# Autodesk Inventor assembly: LightBracketAssembly
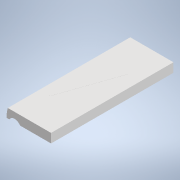
[picture p0: Inventor's stored thumbnail of the model, 180x180]
Saved by Autodesk Inventor 2021.2 (Build 252289000, 289)
## iProperties
Created: 2021-02-05
Part Number: LightBracketAssembly
Document SubType Name: Assembly
Designer: robst
Author: robst
## Documents named in this file (3)
- C:\git\CAD-Development\robSteele\HouseProjects\TrailerProjects\LightBracketAssembly.iam
- C:\git\CAD-Development\robSteele\HouseProjects\TrailerProjects\ketchenLightBracketV02-leftSide.ipt
- C:\git\CAD-Development\robSteele\HouseProjects\TrailerProjects\ketchenLightBracketV02-rightSide.ipt
## Components (2 placed, 2 different names)
1. ketchenLightBracketV02-leftSide:1 — Flush:1, Flush:2, Mate:1
2. ketchenLightBracketV02-rightSide:1 — Flush:1, Flush:2, Mate:1
## Relationships (3: Flush 2, Mate 1)
- Flush:1: ketchenLightBracketV02-leftSide:1 ↔ ketchenLightBracketV02-rightSide:1
- Flush:2: ketchenLightBracketV02-leftSide:1 ↔ ketchenLightBracketV02-rightSide:1
- Mate:1: ketchenLightBracketV02-leftSide:1 ↔ ketchenLightBracketV02-rightSide:1
